# Autodesk Inventor assembly: Full
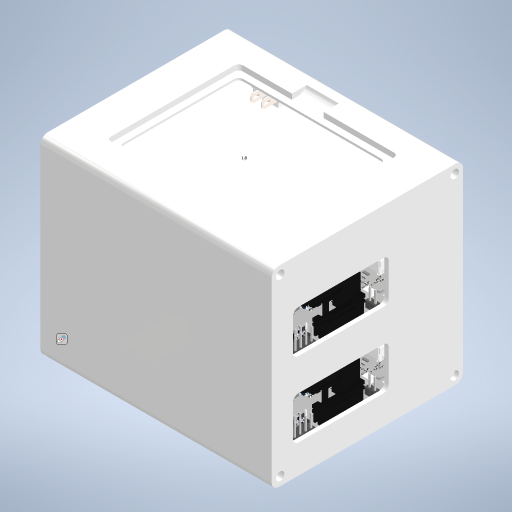
[picture p0: Inventor's stored thumbnail of the model, 512x512]
Saved by Autodesk Inventor 2024 (Build 280153000, 153)
## iProperties
Created: 2023-11-22
Part Number: Full
Document SubType Name: Assembly
Designer: G2O
Author: G2O
## Documents named in this file (6)
- C:\Users\G2O\Documents\Design\Full.iam
- C:\Users\G2O\Documents\Design\Body.ipt
- C:\Users\G2O\Documents\Design\LeftCover.ipt
- C:\Users\G2O\OneDrive - 0bmy3\Dokumentasi TA\Design\Jetson nano 4GB\Jetson nano 4GB.iam
- C:\Users\G2O\OneDrive - 0bmy3\Dokumentasi TA\Design\Switch On_Off\Switch On_Off.ipt
- C:\Users\G2O\Documents\Design\RightCover.ipt
## Components (6 placed, 5 different names)
1. Body:1 — Mate:1, Mate:2, Mate:3, Rigid:1, Cylindrical:1
2. LeftCover:1 — Mate:1
3. Jetson nano 4GB:1 [sub-assembly] — Mate:2
4. Jetson nano 4GB:2 [sub-assembly] — Mate:3
5. Switch On_Off:1 — Rigid:1
6. RightCover:1 — Cylindrical:1
## Relationships (5: Mate 3, WeldJoint 1, CylindricalJoint 1)
- Mate:1: Body:1 ↔ LeftCover:1
- Mate:2: Body:1 ↔ Jetson nano 4GB:1
- Mate:3: Body:1 ↔ Jetson nano 4GB:2
- Rigid:1 [WeldJoint]: Body:1 ↔ Switch On_Off:1
- Cylindrical:1: Body:1 ↔ RightCover:1
